# Autodesk Inventor assembly: Piston Support
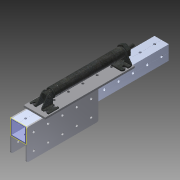
[picture p0: Inventor's stored thumbnail of the model, 180x180]
Saved by Autodesk Inventor 2014 (Build 180170000, 170)
## iProperties
Created: 2014-01-07
Part Number: Piston Support
Document SubType Name: Assembly
Designer: Michael
Author: Michael
## Documents named in this file (5)
- C:\Users\Michael\Documents\GitHub\2014buildCAD\Funnel Catcher\Piston Support.iam
- C:\Users\Michael\Documents\GitHub\2014buildCAD\Funnel Catcher\Support for Connect Arm to Funnel  (Custom).ipt
- C:\Users\Michael\Documents\GitHub\2014buildCAD\Funnel Catcher\9-16 in Pneumatic Cylinder (3 in Stroke).iam
- C:\Users\Michael\Documents\GitHub\2014buildCAD\Funnel Catcher\Vex Pro 1x1 rectangular tubing 7 in length.ipt
- C:\Users\Michael\Documents\GitHub\2014buildCAD\Funnel Catcher\Support for 9-16 Piston.ipt
## Components (5 placed, 4 different names)
1. Support for Connect Arm to Funnel  (Custom):1
2. Support for Connect Arm to Funnel  (Custom):2
3. 9-16 in Pneumatic Cylinder (3 in Stroke):1 [sub-assembly]
4. Vex Pro 1x1 rectangular tubing 7 in length:1
5. Support for 9-16 Piston:1
## Relationships (8: Insert 8)
- [Insert]: 9-16 in Pneumatic Cylinder (3 in Stroke):1 ↔ Support for 9-16 Piston:1
- [Insert]: 9-16 in Pneumatic Cylinder (3 in Stroke):1 ↔ Support for 9-16 Piston:1
- [Insert]: Support for Connect Arm to Funnel  (Custom):2 ↔ Vex Pro 1x1 rectangular tubing 7 in length:1
- [Insert]: Support for Connect Arm to Funnel  (Custom):2 ↔ Vex Pro 1x1 rectangular tubing 7 in length:1
- [Insert]: Support for Connect Arm to Funnel  (Custom):1 ↔ Vex Pro 1x1 rectangular tubing 7 in length:1
- [Insert]: Support for Connect Arm to Funnel  (Custom):1 ↔ Vex Pro 1x1 rectangular tubing 7 in length:1
- [Insert]: Vex Pro 1x1 rectangular tubing 7 in length:1 ↔ Support for 9-16 Piston:1
- [Insert]: Vex Pro 1x1 rectangular tubing 7 in length:1 ↔ Support for 9-16 Piston:1
